# Autodesk Inventor assembly: Base Assembly
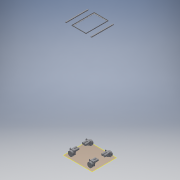
[picture p0: Inventor's stored thumbnail of the model, 180x180]
Saved by Autodesk Inventor 2016 SP2 (Build 200236200, 236)
## iProperties
Created: 2018-01-20
Part Number: Base Assembly
Document SubType Name: Assembly
Designer: CAD
Author: CAD
## Documents named in this file (8)
- C:\Users\CAD\Documents\GitHub\FIRST-ROBOTICS-2018-5436-CAD\Robot\Chassis\Base Assembly.iam
- C:\Users\CAD\Documents\GitHub\FIRST-ROBOTICS-2018-5436-CAD\Robot\Chassis\Gutted Transmission (smaller weight on CAD).iam
- C:\Users\CAD\Documents\GitHub\FIRST-ROBOTICS-2018-5436-CAD\Robot\Chassis\Transmission bracket.ipt
- C:\Users\CAD\Documents\GitHub\FIRST-ROBOTICS-2018-5436-CAD\Robot\Chassis\27.5 L.ipt
- C:\Users\CAD\Documents\GitHub\FIRST-ROBOTICS-2018-5436-CAD\Robot\Climbing Pieces\drive motor + trasmission pieces\Collar.ipt
- C:\Users\CAD\Documents\GitHub\FIRST-ROBOTICS-2018-5436-CAD\Robot\Chassis\Temp Wheels.ipt
- C:\Users\CAD\Documents\GitHub\FIRST-ROBOTICS-2018-5436-CAD\Robot\Chassis\27 in sq frame.ipt
- C:\Users\CAD\Documents\GitHub\FIRST-ROBOTICS-2018-5436-CAD\Robot\Chassis\17.25 L.ipt
## Components (26 placed, 7 different names)
1. Gutted Transmission (smaller weight on CAD):1 [sub-assembly] — Flush:5, Mate:19, Mate:20, Mate:21, Mate:22, Mate:23, Mate:24, Mate:33, Mate:34, Mate:35, Mate:48, Mate:49
2. Gutted Transmission (smaller weight on CAD):2 [sub-assembly] — Mate:13, Mate:14, Mate:15, Mate:16, Mate:17, Mate:18, Flush:3, Mate:30, Mate:31, Mate:32, Mate:45, Mate:46
3. Gutted Transmission (smaller weight on CAD):3 [sub-assembly] — Mate:7, Mate:8, Mate:9, Mate:10, Mate:11, Mate:12, Mate:36, Mate:37, Mate:38, Mate:42, Mate:43, Flush:8
4. Gutted Transmission (smaller weight on CAD):4 [sub-assembly] — Mate:1, Mate:2, Mate:3, Mate:4, Mate:5, Mate:6, Flush:3, Flush:5, Mate:27, Mate:28, Mate:29, Mate:39, Mate:40, Flush:8
5. Transmission bracket:1 — Mate:19, Mate:23, Mate:24, Mate:55
6. Transmission bracket:2 — Mate:20, Mate:21, Mate:22, Flush:10, Mate:57, Mate:68
7. Transmission bracket:3 — Mate:16, Mate:17, Mate:18, Mate:54
8. Transmission bracket:4 — Mate:13, Mate:14, Mate:15, Flush:9, Mate:56, Mate:67
9. Transmission bracket:5 — Mate:10, Mate:11, Mate:12, Mate:52, Flush:10, Mate:69
10. Transmission bracket:6 — Mate:4, Mate:5, Mate:6, Mate:51, Flush:9, Mate:66
11. Transmission bracket:7 — Mate:7, Mate:8, Mate:9
12. Transmission bracket:8 — Mate:1, Mate:2, Mate:3, Mate:25
13. 27.5 L:2 — Mate:25, Flush:6, Flush:7, Mate:52, Flush:11, Mate:59, Mate:62, Flush:13, Mate:63, Mate:69
14. Collar:1 — Mate:30, Mate:31, Mate:32, Mate:47
15. Collar:2 — Mate:33, Mate:34, Mate:35, Mate:50
16. Collar:3 — Mate:27, Mate:28, Mate:29, Mate:41
17. Collar:4 — Mate:36, Mate:37, Mate:38, Mate:44
18. Temp Wheels:1 — Mate:39, Mate:40, Mate:41, Tangent:1
19. Temp Wheels:2 — Mate:42, Mate:43, Mate:44
20. Temp Wheels:3 — Mate:45, Mate:46, Mate:47
21. Temp Wheels:4 — Mate:48, Mate:49, Mate:50
22. 27.5 L:3 — Mate:56, Mate:57, Flush:11, Mate:60, Mate:61, Flush:14, Mate:64, Mate:65, Flush:15, Mate:67, Mate:68
23. 27 in sq frame:1 — Flush:6, Flush:7, Mate:51, Mate:66, Flush:16
24. 27 in sq frame:2 — Mate:54, Mate:55, Angle:1, Flush:14, Flush:16
25. 17.25 L:1 — Mate:59, Mate:60, Mate:61, Mate:62, Flush:13
26. 17.25 L:2 — Mate:63, Mate:64, Mate:65, Flush:15
## Relationships (80: Mate 66, Flush 12, Tangent 1, Angle 1)
- Mate:1: Gutted Transmission (smaller weight on CAD):4 ↔ Transmission bracket:8
- Mate:2: Gutted Transmission (smaller weight on CAD):4 ↔ Transmission bracket:8
- Mate:3: Gutted Transmission (smaller weight on CAD):4 ↔ Transmission bracket:8
- Mate:4: Gutted Transmission (smaller weight on CAD):4 ↔ Transmission bracket:6
- Mate:5: Gutted Transmission (smaller weight on CAD):4 ↔ Transmission bracket:6
- Mate:6: Gutted Transmission (smaller weight on CAD):4 ↔ Transmission bracket:6
- Mate:7: Gutted Transmission (smaller weight on CAD):3 ↔ Transmission bracket:7
- Mate:8: Gutted Transmission (smaller weight on CAD):3 ↔ Transmission bracket:7
- Mate:9: Gutted Transmission (smaller weight on CAD):3 ↔ Transmission bracket:7
- Mate:10: Gutted Transmission (smaller weight on CAD):3 ↔ Transmission bracket:5
- Mate:11: Gutted Transmission (smaller weight on CAD):3 ↔ Transmission bracket:5
- Mate:12: Gutted Transmission (smaller weight on CAD):3 ↔ Transmission bracket:5
- Mate:13: Gutted Transmission (smaller weight on CAD):2 ↔ Transmission bracket:4
- Mate:14: Gutted Transmission (smaller weight on CAD):2 ↔ Transmission bracket:4
- Mate:15: Gutted Transmission (smaller weight on CAD):2 ↔ Transmission bracket:4
- Mate:16: Gutted Transmission (smaller weight on CAD):2 ↔ Transmission bracket:3
- Mate:17: Gutted Transmission (smaller weight on CAD):2 ↔ Transmission bracket:3
- Mate:18: Gutted Transmission (smaller weight on CAD):2 ↔ Transmission bracket:3
- Flush:3: Gutted Transmission (smaller weight on CAD):2 ↔ Gutted Transmission (smaller weight on CAD):4
- Flush:5: Gutted Transmission (smaller weight on CAD):1 ↔ Gutted Transmission (smaller weight on CAD):4
- Mate:19: Gutted Transmission (smaller weight on CAD):1 ↔ Transmission bracket:1
- Mate:20: Gutted Transmission (smaller weight on CAD):1 ↔ Transmission bracket:2
- Mate:21: Gutted Transmission (smaller weight on CAD):1 ↔ Transmission bracket:2
- Mate:22: Gutted Transmission (smaller weight on CAD):1 ↔ Transmission bracket:2
- Mate:23: Gutted Transmission (smaller weight on CAD):1 ↔ Transmission bracket:1
- Mate:24: Gutted Transmission (smaller weight on CAD):1 ↔ Transmission bracket:1
- Mate:25: Transmission bracket:8 ↔ 27.5 L:2
- Mate:27: Gutted Transmission (smaller weight on CAD):4 ↔ Collar:3
- Mate:28: Gutted Transmission (smaller weight on CAD):4 ↔ Collar:3
- Mate:29: Gutted Transmission (smaller weight on CAD):4 ↔ Collar:3
- Mate:30: Gutted Transmission (smaller weight on CAD):2 ↔ Collar:1
- Mate:31: Gutted Transmission (smaller weight on CAD):2 ↔ Collar:1
- Mate:32: Gutted Transmission (smaller weight on CAD):2 ↔ Collar:1
- Mate:33: Gutted Transmission (smaller weight on CAD):1 ↔ Collar:2
- Mate:34: Gutted Transmission (smaller weight on CAD):1 ↔ Collar:2
- Mate:35: Gutted Transmission (smaller weight on CAD):1 ↔ Collar:2
- Mate:36: Gutted Transmission (smaller weight on CAD):3 ↔ Collar:4
- Mate:37: Gutted Transmission (smaller weight on CAD):3 ↔ Collar:4
- Mate:38: Gutted Transmission (smaller weight on CAD):3 ↔ Collar:4
- Mate:39: Gutted Transmission (smaller weight on CAD):4 ↔ Temp Wheels:1
- Mate:40: Gutted Transmission (smaller weight on CAD):4 ↔ Temp Wheels:1
- Mate:41: Collar:3 ↔ Temp Wheels:1
- Mate:42: Gutted Transmission (smaller weight on CAD):3 ↔ Temp Wheels:2
- Mate:43: Gutted Transmission (smaller weight on CAD):3 ↔ Temp Wheels:2
- Mate:44: Collar:4 ↔ Temp Wheels:2
- Mate:45: Gutted Transmission (smaller weight on CAD):2 ↔ Temp Wheels:3
- Mate:46: Gutted Transmission (smaller weight on CAD):2 ↔ Temp Wheels:3
- Mate:47: Collar:1 ↔ Temp Wheels:3
- Mate:48: Gutted Transmission (smaller weight on CAD):1 ↔ Temp Wheels:4
- Mate:49: Gutted Transmission (smaller weight on CAD):1 ↔ Temp Wheels:4
- Mate:50: Collar:2 ↔ Temp Wheels:4
- Flush:6: 27.5 L:2 ↔ 27 in sq frame:1
- Flush:7: 27.5 L:2 ↔ 27 in sq frame:1
- Mate:51: Transmission bracket:6 ↔ 27 in sq frame:1
- Tangent:1: Temp Wheels:1
- Mate:52: Transmission bracket:5 ↔ 27.5 L:2
- Flush:8: Gutted Transmission (smaller weight on CAD):3 ↔ Gutted Transmission (smaller weight on CAD):4
- Mate:54: Transmission bracket:3 ↔ 27 in sq frame:2
- Flush:9: Transmission bracket:4 ↔ Transmission bracket:6
- Flush:10: Transmission bracket:2 ↔ Transmission bracket:5
- Mate:55: Transmission bracket:1 ↔ 27 in sq frame:2
- Mate:56: Transmission bracket:4 ↔ 27.5 L:3
- Mate:57: Transmission bracket:2 ↔ 27.5 L:3
- Flush:11: 27.5 L:2 ↔ 27.5 L:3
- Angle:1 (180 deg): 27 in sq frame:2
- Mate:59: 27.5 L:2 ↔ 17.25 L:1
- Mate:60: 27.5 L:3 ↔ 17.25 L:1
- Mate:61: 27.5 L:3 ↔ 17.25 L:1
- Mate:62: 27.5 L:2 ↔ 17.25 L:1
- Flush:13: 27.5 L:2 ↔ 17.25 L:1
- Flush:14: 27.5 L:3 ↔ 27 in sq frame:2
- Mate:63: 27.5 L:2 ↔ 17.25 L:2
- Mate:64: 27.5 L:3 ↔ 17.25 L:2
- Mate:65: 27.5 L:3 ↔ 17.25 L:2
- Flush:15: 27.5 L:3 ↔ 17.25 L:2
- Mate:66: Transmission bracket:6 ↔ 27 in sq frame:1
- Mate:67: Transmission bracket:4 ↔ 27.5 L:3
- Mate:68: Transmission bracket:2 ↔ 27.5 L:3
- Mate:69: Transmission bracket:5 ↔ 27.5 L:2
- Flush:16: 27 in sq frame:1 ↔ 27 in sq frame:2
